# Autodesk Inventor assembly: Greifer
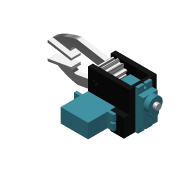
[picture p0: Inventor's stored thumbnail of the model, 180x180]
Saved by Autodesk Inventor 2015 (Build 190159000, 159)
## iProperties
Created: 2015-02-14
Part Number: Greifer
Document SubType Name: Assembly
Designer: Luki
Author: Luki
## Documents named in this file (5)
- C:\Users\Luki\Desktop\Maturaprojekt\Version3\Greifer.iam
- C:\Users\Luki\Desktop\Maturaprojekt\Version3\Greifer1.ipt
- C:\Users\Luki\Desktop\Maturaprojekt\Version3\Greifer2.ipt
- C:\Users\Luki\Desktop\Maturaprojekt\Version3\Greifer3.ipt
- C:\Users\Luki\Desktop\Maturaprojekt\Version3\Mikroservo.ipt
## Components (5 placed, 4 different names)
1. Greifer1:1 — Passend:1, Passend:2, Passend:3, Passend:4, Passend:5, Passend:6, Passend:7, Passend:8, Passend:9, Passend:10, Passend:11, Passend:12, Passend:13
2. Greifer2:1 — Passend:11, Passend:12, Winkel:1, Winkel:2
3. Greifer3:1 — Passend:10, Passend:13, Winkel:1
4. Mikroservo:1 — Passend:7, Passend:8, Passend:9
5. Mikroservo:2 — Passend:4, Passend:5, Passend:6
## Relationships (15: Mate 13, Angle 2)
- Passend:1 [Mate]: Greifer1:1
- Passend:2 [Mate]: Greifer1:1
- Passend:3 [Mate]: Greifer1:1
- Passend:4 [Mate]: Greifer1:1 ↔ Mikroservo:2
- Passend:5 [Mate]: Greifer1:1 ↔ Mikroservo:2
- Passend:6 [Mate]: Greifer1:1 ↔ Mikroservo:2
- Passend:7 [Mate]: Greifer1:1 ↔ Mikroservo:1
- Passend:8 [Mate]: Greifer1:1 ↔ Mikroservo:1
- Passend:9 [Mate]: Greifer1:1 ↔ Mikroservo:1
- Passend:10 [Mate]: Greifer1:1 ↔ Greifer3:1
- Passend:11 [Mate]: Greifer1:1 ↔ Greifer2:1
- Passend:12 [Mate]: Greifer1:1 ↔ Greifer2:1
- Passend:13 [Mate]: Greifer1:1 ↔ Greifer3:1
- Winkel:1 [Angle] (160 deg): Greifer2:1 ↔ Greifer3:1
- Winkel:2 [Angle] (170 deg): Greifer2:1
